# Autodesk Inventor assembly: Hydro400
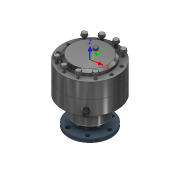
[picture p0: Inventor's stored thumbnail of the model, 180x180]
Saved by Autodesk Inventor 2020.1 (Build 241239000, 239)
## iProperties
Created: 2001-11-10
Part Number: Hydro400
Document SubType Name: Assembly
Designer: Joe M
Engineer: Joe M
Cost Center: 54.288 kg
Authority: 7084887.5 mm^3
Control State: 0
Master: False
Checked Out: False
Shininess: 64.0
Length Units: 11269
Angle Units: 11279
Time Units: 11290
Mass Units: 11283
Length Display Precision: 3
Angle Display Precision: 2
Compacted: True
SaveDate: 2003-11-29
SaveTime: 16:32
TotalMass: 54.288 kg
TotalVolume: 7084887.5 mm^3
Density: 0.0
Volumn: 0.0
Area: 0.0
PropertySet Name: Model Information
Author: Joe M
## Documents named in this file (11)
- C:\Users\thomastremblay\Desktop\Inventor ACP Data\Assemblies\Hydro400.iam
- C:\Users\thomastremblay\Desktop\Inventor ACP Data\Content Center\7055-193.ipt
- C:\Users\thomastremblay\Desktop\Inventor ACP Data\Content Center\7055-191.ipt
- C:\Users\thomastremblay\Desktop\Inventor ACP Data\Content Center\Hardened bush 50x55x20.ipt
- C:\Users\thomastremblay\Desktop\Inventor ACP Data\Content Center\DIN 625 T1 - 6310 - 50 x 110 x 27.ipt
- C:\Users\thomastremblay\Desktop\Inventor ACP Data\Content Center\7055-192.ipt
- C:\Users\thomastremblay\Desktop\Inventor ACP Data\Content Center\DIN 3760 - A - 55 x 72 x 8 - NBR.ipt
- C:\Users\thomastremblay\Desktop\Inventor ACP Data\Assemblies\XL200.iam
- C:\Users\thomastremblay\Desktop\Inventor ACP Data\Content Center\3176 Fitting.ipt
- C:\Users\thomastremblay\Desktop\Inventor ACP Data\Content Center\local.DIN.19.166.1.ipt
- C:\Users\thomastremblay\Desktop\Inventor ACP Data\Content Center\MyStandard.DIN.162.190.1.ipt
## Components (22 placed, 10 different names)
1. 7055-191:1 — Insert:1, Angle:3
2. Hardened bush 50x55x20:1 — Insert:1, Insert:2
3. DIN 625 T1 - 6310 - 50 x 110 x 27:1 — Insert:2, Mate:1, Flush:1
4. DIN 625 T1 - 6310 - 50 x 110 x 27:2 — Insert:5
5. 7055-193:1 — Mate:1, Flush:1, Insert:3, Mate:2, Insert:5, Insert:6, Mate:3, Insert:12, Angle:1, Insert:13, Angle:2
6. 7055-192:1 — Insert:3, Mate:2, Insert:4, Insert:16
7. DIN 3760 - A - 55 x 72 x 8 - NBR:1 — Insert:4
8. XL200:1 [sub-assembly] — Insert:6, Mate:3, Angle:3
9. 3176 Fitting:1 — Insert:12, Angle:1
10. 3176 Fitting:2 — Insert:13, Angle:2
11. DIN 933  (Regelgewinde) - ersetzt durch DIN EN 24 017 M8  x 25:1 — Insert:17
12. DIN 125-1  B B 8.4:1 — Insert:16, Insert:17
13. DIN 933  (Regelgewinde) - ersetzt durch DIN EN 24 017 M8  x 25:2
14. DIN 125-1  B B 8.4:2
15. DIN 933  (Regelgewinde) - ersetzt durch DIN EN 24 017 M8  x 25:3
16. DIN 125-1  B B 8.4:3
17. DIN 933  (Regelgewinde) - ersetzt durch DIN EN 24 017 M8  x 25:4
18. DIN 125-1  B B 8.4:4
19. DIN 933  (Regelgewinde) - ersetzt durch DIN EN 24 017 M8  x 25:5
20. DIN 125-1  B B 8.4:5
21. DIN 933  (Regelgewinde) - ersetzt durch DIN EN 24 017 M8  x 25:6
22. DIN 125-1  B B 8.4:6
## Component patterns: (6 elements, first: DIN 933  (Regelgewinde) - ersetzt durch DIN EN 24 017 M8  x 25:1 + DIN 125-1  B B 8.4:1)
## Relationships (17: Insert 10, Mate 3, Angle 3, Flush 1)
- Insert:1: 7055-191:1 ↔ Hardened bush 50x55x20:1
- Insert:2: Hardened bush 50x55x20:1 ↔ DIN 625 T1 - 6310 - 50 x 110 x 27:1
- Mate:1: DIN 625 T1 - 6310 - 50 x 110 x 27:1 ↔ 7055-193:1
- Flush:1: DIN 625 T1 - 6310 - 50 x 110 x 27:1 ↔ 7055-193:1
- Insert:3: 7055-193:1 ↔ 7055-192:1
- Mate:2: 7055-193:1 ↔ 7055-192:1
- Insert:4: 7055-192:1 ↔ DIN 3760 - A - 55 x 72 x 8 - NBR:1
- Insert:5: DIN 625 T1 - 6310 - 50 x 110 x 27:2 ↔ 7055-193:1
- Insert:6: 7055-193:1 ↔ XL200:1
- Mate:3: 7055-193:1 ↔ XL200:1
- Insert:12: 7055-193:1 ↔ 3176 Fitting:1
- Angle:1 (0 deg): 7055-193:1 ↔ 3176 Fitting:1
- Insert:13: 7055-193:1 ↔ 3176 Fitting:2
- Angle:2 (0 deg): 7055-193:1 ↔ 3176 Fitting:2
- Angle:3 (30 deg): 7055-191:1 ↔ XL200:1
- Insert:16: 7055-192:1 ↔ DIN 125-1  B B 8.4:1
- Insert:17 (-25 mm): DIN 933  (Regelgewinde) - ersetzt durch DIN EN 24 017 M8  x 25:1 ↔ DIN 125-1  B B 8.4:1
